# Autodesk Inventor assembly: green-house
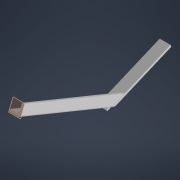
[picture p0: Inventor's stored thumbnail of the model, 180x180]
Saved by Autodesk Inventor 2021 (Build 250183000, 183)
## iProperties
Created: 2020-05-07
Part Number: green-house
Document SubType Name: Assembly
Designer: Jonathan
Author: Jonathan
## Documents named in this file (3)
- C:\Users\Jonathan\green-house\green-house.iam
- C:\Users\Jonathan\green-house\frame.ipt
- C:\Users\Jonathan\green-house\frame-roof.ipt
## Components (2 placed, 2 different names)
1. frame:1 — Mate:1, Mate:2, Mate:3
2. frame-roof:1 — Mate:1, Mate:2, Mate:3
## Relationships (3: Mate 3)
- Mate:1: frame:1 ↔ frame-roof:1
- Mate:2: frame:1 ↔ frame-roof:1
- Mate:3 (0.5 mm): frame:1 ↔ frame-roof:1
